# Autodesk Inventor assembly: Optics Assembly
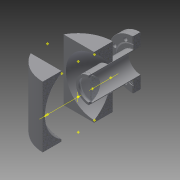
[picture p0: Inventor's stored thumbnail of the model, 180x180]
Saved by Autodesk Inventor 2015 (Build 190159000, 159)
## iProperties
Created: 2014-07-17
Part Number: Optics Assembly
Document SubType Name: Assembly
Designer: I Rabey
Author: I Rabey
## Documents named in this file (5)
- C:\ColdMatter\CADFiles\EDM Machine\Microwave Detection Region\Re-entrant Flange\Optics Assembly.iam
- C:\ColdMatter\CADFiles\EDM Machine\Microwave Detection Region\Re-entrant Flange\Mirror Assembly.iam
- C:\ColdMatter\CADFiles\EDM Machine\Microwave Detection Region\Re-entrant Flange\Re-entrant Flange.iam
- C:\ColdMatter\CADFiles\EDM Machine\Microwave Detection Region\Re-entrant Flange\Custom Mirror Design.ipt
- C:\ColdMatter\CADFiles\EDM Machine\Microwave Detection Region\Re-entrant Flange\Custom Mirror Design Part 2.ipt
## Components (4 placed, 4 different names)
1. Mirror Assembly:1 [sub-assembly]
2. Re-entrant Flange:1 [sub-assembly] — Mate:20, Mate:21, Mate:22, Mate:25
3. Custom Mirror Design:1 — Mate:24, Mate:25
4. Custom Mirror Design Part 2:1 — Mate:21, Mate:23, Mate:24
## Relationships (9: Mate 9)
- Mate:11
- Mate:12
- Mate:19
- Mate:20: Re-entrant Flange:1
- Mate:21: Re-entrant Flange:1 ↔ Custom Mirror Design Part 2:1
- Mate:22 (-32 mm): Re-entrant Flange:1
- Mate:23 (-75 mm): Custom Mirror Design Part 2:1
- Mate:24 (75 mm): Custom Mirror Design:1 ↔ Custom Mirror Design Part 2:1
- Mate:25: Re-entrant Flange:1 ↔ Custom Mirror Design:1
